# Autodesk Inventor assembly: MicroPlast-MB-BG
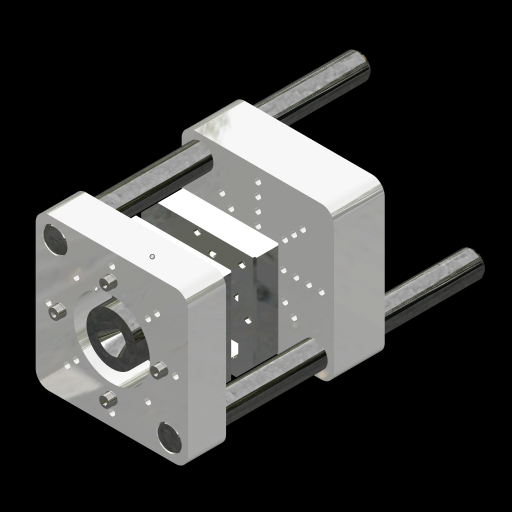
[picture p0: Inventor's stored thumbnail of the model, 512x512]
Saved by Autodesk Inventor 2024 (Build 280153000, 153)
## iProperties
Created: 2023-06-29
Part Number: MicroPlast-MB-BG
Document SubType Name: Assembly
Designer: buchmannmartin
Mass: 4410.95 g
Surface Area: 2254.88 cm^2
Volume: 1292.65 cm^3
Density: 3.41234 g/cm^3
Author: buchmannmartin
## Documents named in this file (12)
- E:\User\Dokumente\#BeneEspressoscope\MicroPlast-MB-BG.iam
- E:\User\Dokumente\#BeneEspressoscope\MP-nozzle.ipt
- E:\User\Dokumente\#BeneEspressoscope\MP-guidance.ipt
- E:\User\Dokumente\#BeneEspressoscope\MP-plate not movable.ipt
- E:\User\Dokumente\#BeneEspressoscope\MP-plate movable.ipt
- E:\User\Dokumente\#BeneEspressoscope\MP-pusher plate.ipt
- E:\User\Dokumente\#BeneEspressoscope\MP-Anschlussfläche.ipt
- E:\User\Dokumente\#BeneEspressoscope\MP-pusher mount.ipt
- E:\User\Dokumente\#BeneEspressoscope\MP-Mould Mount.ipt
- E:\User\Dokumente\Inventor\Content Center Files\R2024\de-DE\ISO 7092\ISO 7092 - ST 5 - 140 HV.ipt
- E:\User\Dokumente\Inventor\Content Center Files\R2024\de-DE\ISO 4762(2)\ISO 4762 - M5 x 50ISO.ipt
- E:\User\Dokumente\#BeneEspressoscope\MP-Mould Mount B.ipt
## Components (17 placed, 11 different names)
1. MP-nozzle:1
2. MP-guidance:1 — Passend:1, Passend:2, Passend:5
3. MP-plate not movable:1 — Passend:3, Passend:4, Fluchtend:2, Fluchtend:3, Passend:6, Passend:7, Passend:8, Passend:9, Passend:10, Passend:11, Passend:12, Passend:13
4. MP-plate movable:1 — Passend:1, Passend:2, Passend:3
5. MP-pusher plate:1 — Passend:4, Fluchtend:1, Passend:5
6. MP-Anschlussfläche:1
7. MP-pusher mount:1 — Fluchtend:2, Fluchtend:3
8. MP-Mould Mount:1 — Fluchtend:4, Fluchtend:5
9. ISO 7092 ST 5 - 140 HV:1 — Passend:6, Passend:7, Einfügen:1
10. ISO 4762 M5 x 50:1 — Einfügen:1
11. MP-Mould Mount B:1 — Fluchtend:4, Fluchtend:5
12. ISO 7092 ST 5 - 140 HV:2 — Passend:8, Passend:9, Einfügen:2
13. ISO 7092 ST 5 - 140 HV:3 — Passend:10, Passend:11, Einfügen:3
14. ISO 7092 ST 5 - 140 HV:4 — Passend:12, Passend:13, Einfügen:4
15. ISO 4762 M5 x 50:2 — Einfügen:2
16. ISO 4762 M5 x 50:3 — Einfügen:3
17. ISO 4762 M5 x 50:4 — Einfügen:4
## Relationships (22: Mate 13, Flush 5, Insert 4)
- Passend:1 [Mate]: MP-guidance:1 ↔ MP-plate movable:1
- Passend:2 [Mate]: MP-guidance:1 ↔ MP-plate movable:1
- Passend:3 [Mate]: MP-plate not movable:1 ↔ MP-plate movable:1
- Passend:4 [Mate]: MP-plate not movable:1 ↔ MP-pusher plate:1
- Fluchtend:1 [Flush]: MP-pusher plate:1
- Passend:5 [Mate]: MP-guidance:1 ↔ MP-pusher plate:1
- Fluchtend:2 [Flush]: MP-plate not movable:1 ↔ MP-pusher mount:1
- Fluchtend:3 [Flush]: MP-plate not movable:1 ↔ MP-pusher mount:1
- Fluchtend:4 [Flush]: MP-Mould Mount:1 ↔ MP-Mould Mount B:1
- Fluchtend:5 [Flush]: MP-Mould Mount:1 ↔ MP-Mould Mount B:1
- Passend:6 [Mate]: MP-plate not movable:1 ↔ ISO 7092 ST 5 - 140 HV:1
- Passend:7 [Mate]: MP-plate not movable:1 ↔ ISO 7092 ST 5 - 140 HV:1
- Passend:8 [Mate]: MP-plate not movable:1 ↔ ISO 7092 ST 5 - 140 HV:2
- Passend:9 [Mate]: MP-plate not movable:1 ↔ ISO 7092 ST 5 - 140 HV:2
- Passend:10 [Mate]: MP-plate not movable:1 ↔ ISO 7092 ST 5 - 140 HV:3
- Passend:11 [Mate]: MP-plate not movable:1 ↔ ISO 7092 ST 5 - 140 HV:3
- Passend:12 [Mate]: MP-plate not movable:1 ↔ ISO 7092 ST 5 - 140 HV:4
- Passend:13 [Mate]: MP-plate not movable:1 ↔ ISO 7092 ST 5 - 140 HV:4
- Einfügen:1 [Insert]: ISO 7092 ST 5 - 140 HV:1 ↔ ISO 4762 M5 x 50:1
- Einfügen:2 [Insert]: ISO 7092 ST 5 - 140 HV:2 ↔ ISO 4762 M5 x 50:2
- Einfügen:3 [Insert]: ISO 7092 ST 5 - 140 HV:3 ↔ ISO 4762 M5 x 50:3
- Einfügen:4 [Insert]: ISO 7092 ST 5 - 140 HV:4 ↔ ISO 4762 M5 x 50:4
